# Autodesk Inventor assembly: FullShortElevator
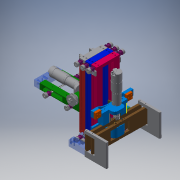
[picture p0: Inventor's stored thumbnail of the model, 180x180]
Saved by Autodesk Inventor 2019 (Build 230136000, 136)
## iProperties
Created: 2019-09-28
Part Number: FullShortElevator
Document SubType Name: Assembly
Designer: james
Author: james
## Documents named in this file (14)
- F:\JimsDesign\Jims2020FTC\FullShortElevator.iam
- F:\JimsDesign\Jims2020FTC\Carrier.iam
- F:\JimsDesign\Jims2020FTC\BackTopBeams.ipt
- F:\JimsDesign\Jims2020FTC\FullElevatorShart.iam
- F:\JimsDesign\Jims2020FTC\ElevDriveShaft.iam
- F:\JimsDesign\Library\ServoCity\5202-0002-0071 part.ipt
- F:\JimsDesign\Library\ServoCity\545548 assembly.iam
- F:\JimsDesign\Library\ServoCity\615460.ipt
- F:\JimsDesign\Library\ServoCity\615456 assembly.iam
- F:\JimsDesign\Jims2020FTC\BackEndSlider.ipt
- F:\JimsDesign\Jims2020FTC\SliderMotorMount.ipt
- F:\JimsDesign\Jims2020FTC\ElevShortBackFrame.iam
- F:\JimsDesign\Jims2020FTC\EvelShortMidFrame.iam
- F:\JimsDesign\Jims2020FTC\EvelShortFrontFrame.iam
## Components (15 placed, 13 different names)
1. ElevShortBackFrame:1 [sub-assembly] — Mate:60, Mate:61, Flush:9, Mate:62, Flush:10
2. EvelShortMidFrame:1 [sub-assembly] — Mate:62, Flush:10, Mate:63, Flush:11
3. EvelShortFrontFrame:1 [sub-assembly] — Mate:63, Flush:11, Mate:64, Flush:12
4. BackTopBeams:1 — Flush:4, Mate:23, Mate:25, Flush:5, Flush:6, Mate:35, Mate:36, Mate:37, Mate:46, Mate:49, Mate:50
5. BackTopBeams:2 — Flush:4, Flush:5, Flush:6, Mate:44, Mate:45, Mate:51, Mate:60, Mate:61, Flush:9
6. FullElevatorShart:1 [sub-assembly] — Mate:25, Mate:37
7. FullElevatorShart:3 [sub-assembly] — Mate:23
8. ElevDriveShaft:1 [sub-assembly] — Mate:35, Mate:36, Mate:40, Mate:41
9. 5202-0002-0071 part:1 — Mate:42, Flush:8, Mate:52, Mate:53
10. Carrier:1 [sub-assembly] — Mate:64, Flush:12
11. 545548 assembly:1 [sub-assembly] — Mate:38, Mate:40
12. 615460:1 — Mate:38, Mate:41
13. 615456 assembly:1 [sub-assembly] — Mate:42, Flush:8
14. BackEndSlider:1 — Mate:44, Mate:45, Mate:46
15. SliderMotorMount:1 — Mate:49, Mate:50, Mate:51, Mate:52, Mate:53
## Relationships (30: Mate 22, Flush 8)
- Flush:4: BackTopBeams:1 ↔ BackTopBeams:2
- Mate:23: BackTopBeams:1 ↔ FullElevatorShart:3
- Mate:25: BackTopBeams:1 ↔ FullElevatorShart:1
- Flush:5: BackTopBeams:1 ↔ BackTopBeams:2
- Flush:6: BackTopBeams:1 ↔ BackTopBeams:2
- Mate:35: BackTopBeams:1 ↔ ElevDriveShaft:1
- Mate:36: BackTopBeams:1 ↔ ElevDriveShaft:1
- Mate:37: BackTopBeams:1 ↔ FullElevatorShart:1
- Mate:38: 545548 assembly:1 ↔ 615460:1
- Mate:40: ElevDriveShaft:1 ↔ 545548 assembly:1
- Mate:41: ElevDriveShaft:1 ↔ 615460:1
- Mate:42: 5202-0002-0071 part:1 ↔ 615456 assembly:1
- Flush:8: 5202-0002-0071 part:1 ↔ 615456 assembly:1
- Mate:44: BackTopBeams:2 ↔ BackEndSlider:1
- Mate:45: BackTopBeams:2 ↔ BackEndSlider:1
- Mate:46: BackTopBeams:1 ↔ BackEndSlider:1
- Mate:49: BackTopBeams:1 ↔ SliderMotorMount:1
- Mate:50: BackTopBeams:1 ↔ SliderMotorMount:1
- Mate:51: BackTopBeams:2 ↔ SliderMotorMount:1
- Mate:52: 5202-0002-0071 part:1 ↔ SliderMotorMount:1
- Mate:53: 5202-0002-0071 part:1 ↔ SliderMotorMount:1
- Mate:60: ElevShortBackFrame:1 ↔ BackTopBeams:2
- Mate:61: ElevShortBackFrame:1 ↔ BackTopBeams:2
- Flush:9: ElevShortBackFrame:1 ↔ BackTopBeams:2
- Mate:62: ElevShortBackFrame:1 ↔ EvelShortMidFrame:1
- Flush:10: ElevShortBackFrame:1 ↔ EvelShortMidFrame:1
- Mate:63: EvelShortMidFrame:1 ↔ EvelShortFrontFrame:1
- Flush:11: EvelShortMidFrame:1 ↔ EvelShortFrontFrame:1
- Mate:64: EvelShortFrontFrame:1 ↔ Carrier:1
- Flush:12: EvelShortFrontFrame:1 ↔ Carrier:1
